# Autodesk Inventor assembly: boitier
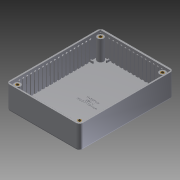
[picture p0: Inventor's stored thumbnail of the model, 180x180]
Saved by Autodesk Inventor 2013 (Build 170138000, 138)
## iProperties
Created: 2013-04-17
Part Number: boitier
Document SubType Name: Assembly
Designer: dimercur
Author: dimercur
## Documents named in this file (3)
- U:\Altium\Ada4Arm\Meca\boitier.iam
- U:\Altium\Ada4Arm\Meca\1591G Box.ipt
- U:\Altium\Ada4Arm\Meca\Insert.ipt
## Components (5 placed, 2 different names)
1. 1591G Box:1 — Placage:1, Placage:2, Placage:3, Placage:4, Affleurement:1, Affleurement:2, Affleurement:3, Affleurement:4
2. Insert:1 — Placage:1, Affleurement:1
3. Insert:2 — Placage:4, Affleurement:2
4. Insert:3 — Placage:3, Affleurement:3
5. Insert:4 — Placage:2, Affleurement:4
## Relationships (8: Mate 4, Flush 4)
- Placage:1 [Mate]: 1591G Box:1 ↔ Insert:1
- Placage:2 [Mate]: 1591G Box:1 ↔ Insert:4
- Placage:3 [Mate]: 1591G Box:1 ↔ Insert:3
- Placage:4 [Mate]: 1591G Box:1 ↔ Insert:2
- Affleurement:1 [Flush]: 1591G Box:1 ↔ Insert:1
- Affleurement:2 [Flush]: 1591G Box:1 ↔ Insert:2
- Affleurement:3 [Flush]: 1591G Box:1 ↔ Insert:3
- Affleurement:4 [Flush]: 1591G Box:1 ↔ Insert:4
